# Autodesk Inventor assembly: GPS_tracker
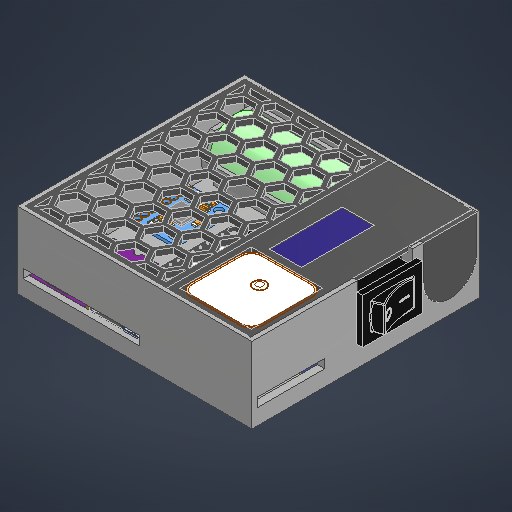
[picture p0: Inventor's stored thumbnail of the model, 512x512]
Saved by Autodesk Inventor 2026.1 (Build 301233020, 233B)
## iProperties
Created: 2026-01-08
Part Number: GPS_tracker
Document SubType Name: Assembly
Designer: Paweł
Author: Paweł
## Documents named in this file (15)
- C:\Users\Paweł\OneDrive - Politechnika Warszawska\Dokumenty\gpstracker\GPS_tracker.iam
- C:\Users\Paweł\OneDrive - Politechnika Warszawska\Dokumenty\gpstracker\pudelko.ipt
- C:\Users\Paweł\OneDrive - Politechnika Warszawska\Dokumenty\gpstracker\Generic Li Ion 1850 cell\18650_cell v1.ipt
- C:\Users\Paweł\OneDrive - Politechnika Warszawska\Dokumenty\gpstracker\ESP-32_v1\ESP-32_v1.iam
- C:\Users\Paweł\OneDrive - Politechnika Warszawska\Dokumenty\gpstracker\GY-NEO6MV2-withAnt v7\A_GPS_ant v2.iam
- C:\Users\Paweł\OneDrive - Politechnika Warszawska\Dokumenty\gpstracker\GY-NEO6MV2-withAnt v7\GPS_ublox_board.iam
- C:\Users\Paweł\OneDrive - Politechnika Warszawska\Dokumenty\gpstracker\MicroSD Card Module - 1\MicroSD Card Module - 1.iam
- C:\Users\Paweł\OneDrive - Politechnika Warszawska\Dokumenty\gpstracker\honneypattern.ipt
- C:\Users\Paweł\OneDrive - Politechnika Warszawska\Dokumenty\gpstracker\ip2368 v5.ipt
- C:\Users\Paweł\OneDrive - Politechnika Warszawska\Dokumenty\gpstracker\klapka.ipt
- C:\Users\Paweł\OneDrive - Politechnika Warszawska\Dokumenty\gpstracker\MPU6050 v2.ipt
- C:\Users\Paweł\OneDrive - Politechnika Warszawska\Dokumenty\gpstracker\pokrywka2.ipt
- C:\Users\Paweł\OneDrive - Politechnika Warszawska\Dokumenty\gpstracker\usbc.ipt
- C:\Users\Paweł\OneDrive - Politechnika Warszawska\Dokumenty\gpstracker\switch 15E20.ipt
- C:\Users\Paweł\OneDrive - Politechnika Warszawska\Dokumenty\gpstracker\OSSD-128x64.ipt
## Components (14 placed, 14 different names)
1. pudelko:1 — Insert:1, Mate:1, Mate:2, Mate:3, Mate:4, Mate:6, Mate:8, Mate:9, Mate:10, Mate:11, Mate:12, Mate:13, Mate:14, Mate:15, Mate:17, Flush:3, Mate:18, Mate:21, Mate:22, Mate:23, Mate:24, Mate:25, Flush:4, Mate:26, Mate:29, Mate:30, Mate:31
2. 18650_cell v1:1 — Insert:1
3. ESP-32_v1:1 [sub-assembly] — Mate:1, Mate:5, Mate:9
4. A_GPS_ant v2:1 [sub-assembly] — Mate:27, Flush:5, Mate:28
5. GPS_ublox_board:1 [sub-assembly] — Mate:6, Mate:7, Mate:8
6. MicroSD Card Module - 1:1 [sub-assembly] — Mate:2, Mate:3, Mate:4, Mate:5, Mate:7
7. honneypattern:1 — Mate:21, Mate:22, Mate:23
8. ip2368 v5:1 — Mate:13, Mate:14, Mate:15, Mate:16, Flush:1, Flush:2
9. klapka:1 — Mate:24, Mate:25, Flush:4, Mate:26
10. MPU6050 v2:1 — Mate:10, Mate:11, Mate:12
11. pokrywka2:1 — Mate:17, Flush:3, Mate:18, Mate:27, Flush:5, Mate:28, Mate:32, Mate:33
12. usbc:1 — Mate:16, Flush:1, Flush:2
13. switch 15E20:1 — Mate:29, Mate:30, Mate:31
14. OSSD-128x64:1 — Mate:32, Mate:33
## Relationships (37: Mate 31, Flush 5, Insert 1)
- Insert:1: pudelko:1 ↔ 18650_cell v1:1
- Mate:1: pudelko:1 ↔ ESP-32_v1:1
- Mate:2: pudelko:1 ↔ MicroSD Card Module - 1:1
- Mate:3: pudelko:1 ↔ MicroSD Card Module - 1:1
- Mate:4 (2 mm): pudelko:1 ↔ MicroSD Card Module - 1:1
- Mate:5 (5 mm): ESP-32_v1:1 ↔ MicroSD Card Module - 1:1
- Mate:6: pudelko:1 ↔ GPS_ublox_board:1
- Mate:7: GPS_ublox_board:1 ↔ MicroSD Card Module - 1:1
- Mate:8 (1 mm): pudelko:1 ↔ GPS_ublox_board:1
- Mate:9: pudelko:1 ↔ ESP-32_v1:1
- Mate:10: pudelko:1 ↔ MPU6050 v2:1
- Mate:11: pudelko:1 ↔ MPU6050 v2:1
- Mate:12 (5 mm): pudelko:1 ↔ MPU6050 v2:1
- Mate:13: pudelko:1 ↔ ip2368 v5:1
- Mate:14: pudelko:1 ↔ ip2368 v5:1
- Mate:15: pudelko:1 ↔ ip2368 v5:1
- Mate:16: ip2368 v5:1 ↔ usbc:1
- Flush:1: ip2368 v5:1 ↔ usbc:1
- Flush:2 (5 mm): ip2368 v5:1 ↔ usbc:1
- Mate:17: pudelko:1 ↔ pokrywka2:1
- Flush:3: pudelko:1 ↔ pokrywka2:1
- Mate:18: pudelko:1 ↔ pokrywka2:1
- Mate:21: pudelko:1 ↔ honneypattern:1
- Mate:22: pudelko:1 ↔ honneypattern:1
- Mate:23: pudelko:1 ↔ honneypattern:1
- Mate:24: pudelko:1 ↔ klapka:1
- Mate:25: pudelko:1 ↔ klapka:1
- Flush:4: pudelko:1 ↔ klapka:1
- Mate:26: pudelko:1 ↔ klapka:1
- Mate:27: A_GPS_ant v2:1 ↔ pokrywka2:1
- Flush:5: A_GPS_ant v2:1 ↔ pokrywka2:1
- Mate:28: A_GPS_ant v2:1 ↔ pokrywka2:1
- Mate:29: pudelko:1 ↔ switch 15E20:1
- Mate:30: pudelko:1 ↔ switch 15E20:1
- Mate:31: pudelko:1 ↔ switch 15E20:1
- Mate:32: pokrywka2:1 ↔ OSSD-128x64:1
- Mate:33: pokrywka2:1 ↔ OSSD-128x64:1
